# Autodesk Inventor assembly: Übertragung des Zahnriemens
Saved by Autodesk Inventor 2016 (Build 200138000, 138)
## iProperties
Created: 2015-08-10
Part Number: Übertragung des Zahnriemens
Document SubType Name: Assembly
Designer: 4ndreas
ClientObjectVersion: 1
Author: 4ndreas
## Documents named in this file (5)
- C:\Users\4ndreas\Documents\Inventor\RobotARM v2\v4\StepperBase\Konstruktions-Assistent\Übertragung des Zahnriemens1.iam
- C:\Users\4ndreas\Documents\Inventor\RobotARM v2\v4\StepperBase\Konstruktions-Assistent\Zahnriemen1.ipt
- C:\Users\4ndreas\Documents\Inventor\RobotARM v2\v4\StepperBase\Konstruktions-Assistent\Flache Riemenscheibe21.ipt
- C:\Users\4ndreas\Documents\Inventor\RobotARM v2\v4\StepperBase\Konstruktions-Assistent\Synchrone Riemenscheibe21.ipt
- C:\Users\4ndreas\Documents\Inventor\RobotARM v2\v4\StepperBase\Konstruktions-Assistent\Flache Riemenscheibe11.ipt
## Components (4 placed, 4 different names)
1. Zahnriemen:1 — Fluchtend:1, Passend:1, Fluchtend:2, Passend:2, Passend:3, Fluchtend:3, Passend:4
2. Flache Riemenscheibe2:1 — Fluchtend:1, Passend:1
3. Synchrone Riemenscheibe2:1 — Fluchtend:2, Passend:2, Passend:3
4. Flache Riemenscheibe1:1 — Fluchtend:3, Passend:4
## Relationships (7: Mate 4, Flush 3)
- Fluchtend:1 [Flush]: Zahnriemen:1 ↔ Flache Riemenscheibe2:1
- Passend:1 [Mate]: Zahnriemen:1 ↔ Flache Riemenscheibe2:1
- Fluchtend:2 [Flush]: Zahnriemen:1 ↔ Synchrone Riemenscheibe2:1
- Passend:2 [Mate]: Zahnriemen:1 ↔ Synchrone Riemenscheibe2:1
- Passend:3 [Mate]: Zahnriemen:1 ↔ Synchrone Riemenscheibe2:1
- Fluchtend:3 [Flush]: Zahnriemen:1 ↔ Flache Riemenscheibe1:1
- Passend:4 [Mate]: Zahnriemen:1 ↔ Flache Riemenscheibe1:1
